# Autodesk Inventor assembly: AC254-075-OnPost
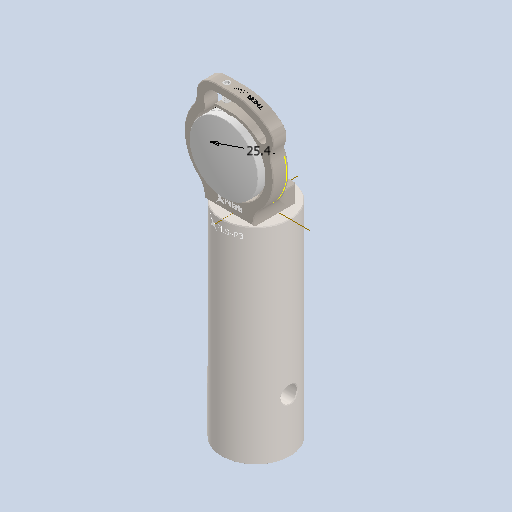
[picture p0: Inventor's stored thumbnail of the model, 512x512]
Saved by Autodesk Inventor 2025.2 (Build 292293000, 293)
## iProperties
Created: 2025-04-04
Part Number: AC254-075-OnPost
Document SubType Name: Assembly
Designer: monolithic
Author: monolithic
## Documents named in this file (3)
- C:\Users\monolithic\Documents\GitHub\CAD\Monolith\John\Altair_PowellBaseplate_SPIM_ASLM_CTASLM\Assembly\SubAssemblies\AC254-075-OnPost.iam
- C:\Users\monolithic\Documents\GitHub\CAD\Monolith\John\Altair_PowellBaseplate_SPIM_ASLM_CTASLM\Assembly\SubAssemblies\PostLensHolder_B1S_PLS3in.iam
- C:\Users\monolithic\Documents\GitHub\CAD\Monolith\John\Altair_PowellBaseplate_SPIM_ASLM_CTASLM\Assembly\SubAssemblies\AC254-075-A-Step.ipt
## Components (2 placed, 2 different names)
1. PostLensHolder_B1S_PLS3in:1 [sub-assembly] — Mate:1, Angle:1, Mate:2, Angle:2
2. AC254-075-A-Step:1 — Mate:1, Tangent:1
## Relationships (5: Mate 2, Angle 2, Tangent 1)
- Mate:1: PostLensHolder_B1S_PLS3in:1 ↔ AC254-075-A-Step:1
- Angle:1 (0 deg): PostLensHolder_B1S_PLS3in:1
- Tangent:1: AC254-075-A-Step:1
- Mate:2: PostLensHolder_B1S_PLS3in:1
- Angle:2 (0 deg): PostLensHolder_B1S_PLS3in:1
